# Autodesk Inventor assembly: FLUGGER CAP TRAY ASSY
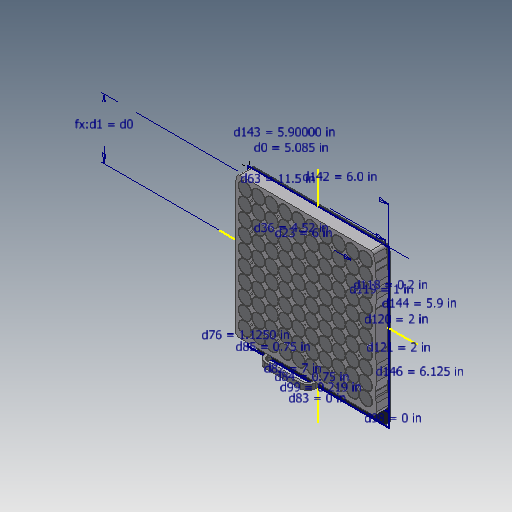
[picture p0: Inventor's stored thumbnail of the model, 512x512]
Saved by Autodesk Inventor 2020.3 (Build 243373000, 373)
## iProperties
RuleStatus: InUse
AfterDocSave0: file://Part Number Cleaner
Created: 2018-10-13
Vendor: HHMI: JRC - ID&F
Document SubType Name: Assembly
Designer: arnoldj
DESIGN DEPARTMENT: HHMI: JRC - ID&F
ALTERED ITEM PART NUMBER: N/A
ALTERED ITEM VENDOR: N/A
ALTERED ITEM DESCRIPTION: N/A
Author: arnoldj
Revision Number: 0
## Documents named in this file (5)
- C:\_WORKSPACE\DATA\PROJECTS\_PROJECTS BY LAB\CARD (LAB)\FLUGGER\FLUGGER CAP TRAY ASSY.iam
- C:\_WORKSPACE\DATA\PROJECTS\_PROJECTS BY LAB\FLY FACILITY\FLY MEDIA VIAL PLUGGING\GENESEE 49-101.ipt
- C:\_WORKSPACE\DATA\COMMON\McMaster\MCMASTER 1855A640_PULL HANDLE.ipt
- C:\_WORKSPACE\DATA\PROJECTS\_PROJECTS BY LAB\FLY FACILITY\FLY MEDIA VIAL PLUGGING\VP CAP LAYER 10x10 V3.ipt
- C:\_WORKSPACE\DATA\PROJECTS\_PROJECTS BY LAB\FLY FACILITY\FLY MEDIA VIAL PLUGGING\VP COMP LAYER H 10x10 V3.ipt
## Components (103 placed, 4 different names)
1. VP COMP LAYER H 10x10 V3:1 — Mate:1, Flush:1, Flush:2, Mate:2, Mate:7, Mate:8, Mate:9
2. VP CAP LAYER 10x10 V3:1 — Mate:1, Flush:1, Flush:2, Mate:3
3. MCMASTER 1855A640_PULL HANDLE:1 — Mate:7, Mate:8, Mate:9
4. GENESEE 49-101:1 — Mate:2, Mate:3
5. GENESEE 49-101:2
6. GENESEE 49-101:3
7. GENESEE 49-101:4
8. GENESEE 49-101:5
9. GENESEE 49-101:6
10. GENESEE 49-101:7
11. GENESEE 49-101:8
12. GENESEE 49-101:9
13. GENESEE 49-101:10
14. GENESEE 49-101:11
15. GENESEE 49-101:12
16. GENESEE 49-101:13
17. GENESEE 49-101:14
18. GENESEE 49-101:15
19. GENESEE 49-101:16
20. GENESEE 49-101:17
21. GENESEE 49-101:18
22. GENESEE 49-101:19
23. GENESEE 49-101:20
24. GENESEE 49-101:21
25. GENESEE 49-101:22
26. GENESEE 49-101:23
27. GENESEE 49-101:24
28. GENESEE 49-101:25
29. GENESEE 49-101:26
30. GENESEE 49-101:27
31. GENESEE 49-101:28
32. GENESEE 49-101:29
33. GENESEE 49-101:30
34. GENESEE 49-101:31
35. GENESEE 49-101:32
36. GENESEE 49-101:33
37. GENESEE 49-101:34
38. GENESEE 49-101:35
39. GENESEE 49-101:36
40. GENESEE 49-101:37
41. GENESEE 49-101:38
42. GENESEE 49-101:39
43. GENESEE 49-101:40
44. GENESEE 49-101:41
45. GENESEE 49-101:42
46. GENESEE 49-101:43
47. GENESEE 49-101:44
48. GENESEE 49-101:45
49. GENESEE 49-101:46
50. GENESEE 49-101:47
51. GENESEE 49-101:48
52. GENESEE 49-101:49
53. GENESEE 49-101:50
54. GENESEE 49-101:51
55. GENESEE 49-101:52
56. GENESEE 49-101:53
57. GENESEE 49-101:54
58. GENESEE 49-101:55
59. GENESEE 49-101:56
60. GENESEE 49-101:57
61. GENESEE 49-101:58
62. GENESEE 49-101:59
63. GENESEE 49-101:60
64. GENESEE 49-101:61
65. GENESEE 49-101:62
66. GENESEE 49-101:63
67. GENESEE 49-101:64
68. GENESEE 49-101:65
69. GENESEE 49-101:66
70. GENESEE 49-101:67
71. GENESEE 49-101:68
72. GENESEE 49-101:69
73. GENESEE 49-101:70
74. GENESEE 49-101:71
75. GENESEE 49-101:72
76. GENESEE 49-101:73
77. GENESEE 49-101:74
78. GENESEE 49-101:75
79. GENESEE 49-101:76
80. GENESEE 49-101:77
81. GENESEE 49-101:78
82. GENESEE 49-101:79
83. GENESEE 49-101:80
84. GENESEE 49-101:81
85. GENESEE 49-101:82
86. GENESEE 49-101:83
87. GENESEE 49-101:84
88. GENESEE 49-101:85
89. GENESEE 49-101:86
90. GENESEE 49-101:87
91. GENESEE 49-101:88
92. GENESEE 49-101:89
93. GENESEE 49-101:90
94. GENESEE 49-101:91
95. GENESEE 49-101:92
96. GENESEE 49-101:93
97. GENESEE 49-101:94
98. GENESEE 49-101:95
99. GENESEE 49-101:96
100. GENESEE 49-101:97
101. GENESEE 49-101:98
102. GENESEE 49-101:99
103. GENESEE 49-101:100
## Component patterns: (100 elements, first: GENESEE 49-101:1)
## Relationships (8: Mate 6, Flush 2)
- Mate:1: VP COMP LAYER H 10x10 V3:1 ↔ VP CAP LAYER 10x10 V3:1
- Flush:1: VP COMP LAYER H 10x10 V3:1 ↔ VP CAP LAYER 10x10 V3:1
- Flush:2: VP COMP LAYER H 10x10 V3:1 ↔ VP CAP LAYER 10x10 V3:1
- Mate:2 (-2.032 mm): VP COMP LAYER H 10x10 V3:1 ↔ GENESEE 49-101:1
- Mate:3: VP CAP LAYER 10x10 V3:1 ↔ GENESEE 49-101:1
- Mate:7: VP COMP LAYER H 10x10 V3:1 ↔ MCMASTER 1855A640_PULL HANDLE:1
- Mate:8: VP COMP LAYER H 10x10 V3:1 ↔ MCMASTER 1855A640_PULL HANDLE:1
- Mate:9: VP COMP LAYER H 10x10 V3:1 ↔ MCMASTER 1855A640_PULL HANDLE:1
